# Autodesk Inventor assembly: 123
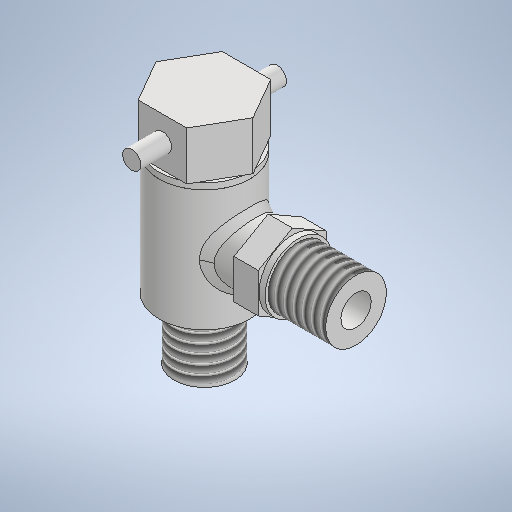
[picture p0: Inventor's stored thumbnail of the model, 512x512]
Saved by Autodesk Inventor 2025.1 (Build 291241000, 241)
## iProperties
Created: 2024-08-22
Part Number: 123
Document SubType Name: Assembly
Designer: ffogue
Author: ffogue
## Documents named in this file (3)
- C:\Projkete - Übungen\Freedom\123.iam
- C:\Projkete - Übungen\Freedom\123.ipt
- C:\Projkete - Übungen\Freedom\123 cap.ipt
## Components (2 placed, 2 different names)
1. 123:1 — Mate:1, Rotational:1
2. 123 cap:1 — Mate:1, Rotational:1
## Relationships (2: Mate 1, RevoluteJoint 1)
- Mate:1: 123:1 ↔ 123 cap:1
- Rotational:1 [RevoluteJoint] (-7 mm): 123:1 ↔ 123 cap:1
